# Autodesk Inventor assembly: assy_gic_kinematic_2d_robot_arm_MK1_v3
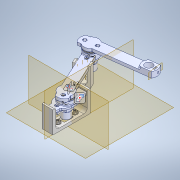
[picture p0: Inventor's stored thumbnail of the model, 180x180]
Saved by Autodesk Inventor 2021 (Build 250183000, 183)
## iProperties
Created: 2021-02-28
Part Number: assy_gic_kinematic_2d_robot_arm_MK1_v3
Document SubType Name: Assembly
Designer: Sam
Author: Sam
## Documents named in this file (11)
- D:\OneDrive\MSc Robotics\GIC\RobotKinematics-Remote\3D CAD\Autodesk\23022021\assy_gic_kinematic_2d_robot_arm_MK1_v3.iam
- D:\OneDrive\MSc Robotics\GIC\RobotKinematics-Remote\3D CAD\Autodesk\23022021\Base_Lower_v3.ipt
- C:\Users\Sam\Documents\Inventor\Content Center Files\R2021\en-US\BS EN ISO 7045 Z\EN ISO 7045 - M5 x 8 - 4.8 - Z(1).ipt
- D:\OneDrive\MSc Robotics\GIC\RobotKinematics-Remote\3D CAD\Autodesk\15012021\DfRobot_stepper_FIT0503_mount_v4.ipt
- D:\OneDrive\MSc Robotics\GIC\RobotKinematics-Remote\3D CAD\Autodesk\15012021\Df_Robot_stepper_FIT0503.ipt
- D:\OneDrive\MSc Robotics\GIC\RobotKinematics-Remote\3D CAD\Autodesk\23022021\base_bearing_holder_v2.ipt
- D:\OneDrive\MSc Robotics\GIC\RobotKinematics-Remote\3D CAD\Autodesk\23022021\608_Z.iam
- D:\OneDrive\MSc Robotics\GIC\RobotKinematics-Remote\3D CAD\Autodesk\23022021\sub_assy_robot_arm_link1.iam
- D:\OneDrive\MSc Robotics\GIC\RobotKinematics-Remote\3D CAD\Autodesk\23022021\sub_assy_robot_arm_link2.iam
- D:\OneDrive\MSc Robotics\GIC\RobotKinematics-Remote\3D CAD\Autodesk\23022021\BallCasterMount.ipt
- D:\OneDrive\MSc Robotics\GIC\RobotKinematics-Remote\3D CAD\Autodesk\23022021\Pololu 1-2in Ball caster.ipt
## Components (11 placed, 10 different names)
1. Base_Lower_v3:1 — Mate:1, Mate:2, Mate:3, Mate:4, Mate:5, Mate:9, Mate:10, Flush:2
2. BS EN ISO 7045 Z - Metric M5 x 8 - 4.8 - Z:1 — Mate:1, Mate:2
3. BS EN ISO 7045 Z - Metric M5 x 8 - 4.8 - Z:2 — Mate:3, Mate:4
4. DfRobot_stepper_FIT0503_mount_v4:1 — Mate:5, Mate:6, Mate:7, Mate:8, Mate:11, Mate:12, Mate:13
5. Df_Robot_stepper_FIT0503:1 — Mate:6, Mate:7, Mate:8
6. base_bearing_holder_v2:1 — Mate:9, Mate:10, Flush:2, Mate:11, Mate:12, Mate:13, Mate:14, Mate:15
7. 608_Z:1 [sub-assembly] — Mate:14, Mate:15, Mate:16, Mate:17, Mate:18
8. sub_assy_robot_arm_link1:1 [sub-assembly] — Mate:16, Mate:17, Mate:18, Mate:19, Mate:20, Mate:21, Mate:22, Flush:3
9. sub_assy_robot_arm_link2:1 [sub-assembly] — Mate:19, Mate:20
10. BallCasterMount:1 — Mate:21, Mate:22, Flush:3, Mate:23, Mate:24, Mate:25
11. Pololu 1-2in Ball caster:1 — Mate:23, Mate:24, Mate:25
## Relationships (27: Mate 25, Flush 2)
- Mate:1: Base_Lower_v3:1 ↔ BS EN ISO 7045 Z - Metric M5 x 8 - 4.8 - Z:1
- Mate:2: Base_Lower_v3:1 ↔ BS EN ISO 7045 Z - Metric M5 x 8 - 4.8 - Z:1
- Mate:3: Base_Lower_v3:1 ↔ BS EN ISO 7045 Z - Metric M5 x 8 - 4.8 - Z:2
- Mate:4: Base_Lower_v3:1 ↔ BS EN ISO 7045 Z - Metric M5 x 8 - 4.8 - Z:2
- Mate:5: Base_Lower_v3:1 ↔ DfRobot_stepper_FIT0503_mount_v4:1
- Mate:6: DfRobot_stepper_FIT0503_mount_v4:1 ↔ Df_Robot_stepper_FIT0503:1
- Mate:7: DfRobot_stepper_FIT0503_mount_v4:1 ↔ Df_Robot_stepper_FIT0503:1
- Mate:8: DfRobot_stepper_FIT0503_mount_v4:1 ↔ Df_Robot_stepper_FIT0503:1
- Mate:9: Base_Lower_v3:1 ↔ base_bearing_holder_v2:1
- Mate:10: Base_Lower_v3:1 ↔ base_bearing_holder_v2:1
- Flush:2: Base_Lower_v3:1 ↔ base_bearing_holder_v2:1
- Mate:11: DfRobot_stepper_FIT0503_mount_v4:1 ↔ base_bearing_holder_v2:1
- Mate:12: DfRobot_stepper_FIT0503_mount_v4:1 ↔ base_bearing_holder_v2:1
- Mate:13: DfRobot_stepper_FIT0503_mount_v4:1 ↔ base_bearing_holder_v2:1
- Mate:14: base_bearing_holder_v2:1 ↔ 608_Z:1
- Mate:15: base_bearing_holder_v2:1 ↔ 608_Z:1
- Mate:16: 608_Z:1 ↔ sub_assy_robot_arm_link1:1
- Mate:17: 608_Z:1 ↔ sub_assy_robot_arm_link1:1
- Mate:18: 608_Z:1 ↔ sub_assy_robot_arm_link1:1
- Mate:19: sub_assy_robot_arm_link1:1 ↔ sub_assy_robot_arm_link2:1
- Mate:20: sub_assy_robot_arm_link1:1 ↔ sub_assy_robot_arm_link2:1
- Mate:21: sub_assy_robot_arm_link1:1 ↔ BallCasterMount:1
- Mate:22: sub_assy_robot_arm_link1:1 ↔ BallCasterMount:1
- Flush:3 (30 mm): sub_assy_robot_arm_link1:1 ↔ BallCasterMount:1
- Mate:23: BallCasterMount:1 ↔ Pololu 1-2in Ball caster:1
- Mate:24: BallCasterMount:1 ↔ Pololu 1-2in Ball caster:1
- Mate:25: BallCasterMount:1 ↔ Pololu 1-2in Ball caster:1
